# Autodesk Inventor assembly: basket_centered
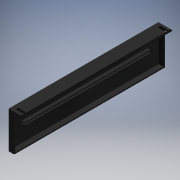
[picture p0: Inventor's stored thumbnail of the model, 180x180]
Saved by Autodesk Inventor 2019.3 (Build 233278000, 278)
## iProperties
Created: 2020-12-03
Part Number: basket_centered
Material: Generisch
Document SubType Name: Assembly
Designer: Nicolas Frick
Mass: 80.6375 g
Surface Area: 498.909 cm^2
Volume: 56.5877 cm^3
Density: 1.425 g/cm^3
Author: Nicolas Frick
## Documents named in this file (2)
- C:\Users\Nicolas Frick\Sync\OneDrive\airhockeybot\mechanical_design\common_cad_parts\sim_models\basket_centered.iam
- C:\Users\Nicolas Frick\Sync\OneDrive\airhockeybot\mechanical_design\inventor\Basket.ipt
## Components (1 placed, 1 different names)
1. Basket:1 — Passend:1, Passend:2, Passend:3
## Relationships (3: Mate 3)
- Passend:1 [Mate]: Basket:1
- Passend:2 [Mate]: Basket:1
- Passend:3 [Mate] (15 mm): Basket:1
